# Autodesk Inventor assembly: Assembly8
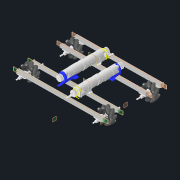
[picture p0: Inventor's stored thumbnail of the model, 180x180]
Saved by Autodesk Inventor 2022 (Build 260153000, 153)
## iProperties
Created: 2021-11-02
Part Number: Assembly8
Document SubType Name: Assembly
Designer: divid
Author: divid
## Documents named in this file (2)
- C:\Users\divid\Documents\GitHub\ComputerAidedDesign\2021-22\FTC\#13822 Robovikes\Drivetrain\Assembly8.iam
- C:\Users\divid\Documents\GitHub\ComputerAidedDesign\2021-22\FTC\#13822 Robovikes\Drivetrain\Drivetrain.iam
## Components (2 placed, 1 different names)
1. Drivetrain:1 [sub-assembly] — Flush:1, Flush:2, Mate:1
2. Drivetrain:2 [sub-assembly] — Flush:1, Flush:2, Mate:1
## Relationships (3: Flush 2, Mate 1)
- Flush:1: Drivetrain:1 ↔ Drivetrain:2
- Flush:2: Drivetrain:1 ↔ Drivetrain:2
- Mate:1 (127 mm): Drivetrain:1 ↔ Drivetrain:2
